# Autodesk Inventor assembly: robot assembly full
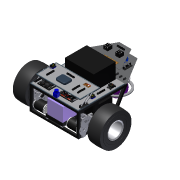
[picture p0: Inventor's stored thumbnail of the model, 180x180]
Saved by Autodesk Inventor 2012 (Build 160160000, 160)
## iProperties
Created: 2011-10-05
Part Number: robot assembly full
Document SubType Name: Assembly
Designer: Antonella
Author: Antonella
## Documents named in this file (5)
- C:\Users\Antonella\Documents\GCC Robotics 2012 - Mechanical\Robot 2.0\robot assembly full.iam
- C:\Users\Antonella\Documents\GCC Robotics 2012 - Mechanical\Robot 2.0\mechanical assembly.iam
- C:\Users\Antonella\Documents\GCC Robotics 2012 - Mechanical\Robot 2.0\Electrical\computer model.ipt
- C:\Users\Antonella\Documents\GCC Robotics 2012 - Mechanical\Robot 2.0\Electrical\Front Electrical Board\Front Electrical Board.iam
- C:\Users\Antonella\Documents\GCC Robotics 2012 - Mechanical\Robot 2.0\Electrical\Back Electrical Board\Back Electrical Board.iam
## Components (4 placed, 4 different names)
1. mechanical assembly:1 [sub-assembly] — Mate:9, Mate:45, Flush:10, Flush:47, Mate:46, Mate:47, Flush:48, Flush:49
2. computer model:1 — Mate:9, Mate:45
3. Front Electrical Board:1 [sub-assembly] — Flush:10, Flush:47, Mate:46
4. Back Electrical Board:1 [sub-assembly] — Mate:47, Flush:48, Flush:49
## Relationships (8: Mate 4, Flush 4)
- Mate:9: mechanical assembly:1 ↔ computer model:1
- Mate:45: mechanical assembly:1 ↔ computer model:1
- Flush:10: mechanical assembly:1 ↔ Front Electrical Board:1
- Flush:47: mechanical assembly:1 ↔ Front Electrical Board:1
- Mate:46: mechanical assembly:1 ↔ Front Electrical Board:1
- Mate:47: mechanical assembly:1 ↔ Back Electrical Board:1
- Flush:48: mechanical assembly:1 ↔ Back Electrical Board:1
- Flush:49: mechanical assembly:1 ↔ Back Electrical Board:1
